# Autodesk Inventor assembly: Final
(part 2 of 3)
475. din1587-m5x0_8ricu3:15 — Mate:506, Mate:512
476. din1587-m5x0_8ricu3:16 — Mate:505, Mate:513
477. din1587-m5x0_8ricu3:17 — Mate:504, Mate:511
478. din1587-m6x1ricu3:3 — Mate:476, Mate:477
## Relationships (1050: Mate 990, Flush 53, Angle 7)
- Flush:1: bottom:1
- Flush:2: bottom:1
- Mate:1: bottom:1
- Mate:2: bottom:1 ↔ SeitenUntenHinten:1
- Mate:3: bottom:1 ↔ SeitenUntenHinten:1
- Mate:4: bottom:1 ↔ SeitenUntenHinten:1
- Mate:8: bottom:1 ↔ Heatsink:1
- Mate:9: bottom:1 ↔ Heatsink:1
- Mate:10: bottom:1 ↔ Heatsink:1
- Mate:11: EndStück_Caps:2 ↔ SeitenUntenHinten:1
- Mate:12: EndStück_Caps:2 ↔ SeitenUntenHinten:1
- Mate:13: EndStück_Caps:2 ↔ SeitenUntenHinten:1
- Mate:14: SeitenUntenHinten:1 ↔ Cap:1
- Mate:15: SeitenUntenHinten:1 ↔ Cap:2
- Mate:16: EndStück_Caps:2 ↔ Cap:2
- Mate:17: EndStück_Caps:2 ↔ Cap:1
- Mate:18: EndStück_Caps:1 ↔ Cap:1
- Mate:19: EndStück_Caps:1 ↔ Cap:1
- Mate:20: EndStück_Caps:1 ↔ Cap:2
- Mate:21: Cap:2 ↔ MidStück_Caps:1
- Mate:22: EndStück_Caps:1 ↔ MidStück_Caps:1
- Mate:23: Cap:1 ↔ MidStück_Caps:1
- Mate:24: SeitenUntenHinten:1 ↔ mid:1
- Mate:25: SeitenUntenHinten:1 ↔ mid:1
- Mate:26: SeitenUntenHinten:1 ↔ mid:1
- Mate:27: bottom:1 ↔ LogicHolder:1
- Mate:28: bottom:1 ↔ LogicHolder:1
- Mate:29: bottom:1 ↔ LogicHolder:1
- Mate:31: Elektronik_Gehäuse:1 ↔ LogicHolder:1
- Mate:32: Elektronik_Gehäuse:1 ↔ LogicHolder:1
- Mate:33: bottom:1 ↔ NtHolder:1
- Mate:36: bottom:1 ↔ SeitenUnten:2
- Mate:37: bottom:1 ↔ SeitenUnten:1
- Mate:38: bottom:1 ↔ SeitenUnten:1
- Mate:39: bottom:1 ↔ SeitenUnten:2
- Mate:40: bottom:1 ↔ SeitenUnten:2
- Mate:41: bottom:1 ↔ SeitenUnten:1
- Mate:42: SeitenUntenVorne:1 ↔ ToslinkHalter:1
- Mate:43: SeitenUntenVorne:1 ↔ ToslinkHalter:1
- Mate:45: Heatsink:1 ↔ GT175DA120U:2
- Mate:46: Heatsink:1 ↔ GT175DA120U:4
- Mate:47: Heatsink:1 ↔ GT175DA120U:3
- Mate:48: Heatsink:1 ↔ GT175DA120U:1
- Mate:49: Heatsink:1 ↔ GT175DA120U:1
- Mate:50: Heatsink:1 ↔ GT175DA120U:1
- Mate:51: Heatsink:1 ↔ GT175DA120U:2
- Mate:52: Heatsink:1 ↔ GT175DA120U:2
- Mate:53: Heatsink:1 ↔ GT175DA120U:4
- Mate:54: Heatsink:1 ↔ GT175DA120U:4
- Mate:55: Heatsink:1 ↔ GT175DA120U:3
- Mate:56: Heatsink:1 ↔ GT175DA120U:3
- Mate:57: IGBT_Platine:3 ↔ GT175DA120U:1
- Mate:58: IGBT_Platine:4 ↔ GT175DA120U:2
- Mate:59: IGBT_Platine:2 ↔ GT175DA120U:3
- Mate:60: IGBT_Platine:1 ↔ GT175DA120U:4
- Mate:61: IGBT_Platine:2 ↔ GT175DA120U:3
- Mate:62: IGBT_Platine:2 ↔ GT175DA120U:3
- Mate:63: IGBT_Platine:1 ↔ GT175DA120U:4
- Mate:64: IGBT_Platine:1 ↔ GT175DA120U:4
- Mate:65: IGBT_Platine:3 ↔ GT175DA120U:1
- Mate:66: IGBT_Platine:3 ↔ GT175DA120U:1
- Mate:67: IGBT_Platine:4 ↔ GT175DA120U:2
- Mate:68: IGBT_Platine:4 ↔ GT175DA120U:2
- Mate:69: IGBT_Platine:1 ↔ din125-1-a_4_3-140_hv:12
- Mate:70: IGBT_Platine:1 ↔ din125-1-a_4_3-140_hv:3
- Mate:71: IGBT_Platine:1 ↔ din125-1-a_4_3-140_hv:4
- Mate:72: IGBT_Platine:1 ↔ din125-1-a_4_3-140_hv:1
- Mate:73: IGBT_Platine:1 ↔ din125-1-a_4_3-140_hv:1
- Mate:74: IGBT_Platine:1 ↔ din125-1-a_4_3-140_hv:12
- Mate:75: IGBT_Platine:1 ↔ din125-1-a_4_3-140_hv:4
- Mate:76: IGBT_Platine:1 ↔ din125-1-a_4_3-140_hv:3
- Mate:77: Abstandshalter_12mm_M4:9 ↔ din125-1-a_4_3-140_hv:1
- Mate:78: Abstandshalter_12mm_M4:1 ↔ din125-1-a_4_3-140_hv:3
- Mate:79: Abstandshalter_12mm_M4:3 ↔ din125-1-a_4_3-140_hv:12
- Mate:80: GT175DA120U:4 ↔ Abstandshalter_12mm_M4:9
- Mate:81: GT175DA120U:4 ↔ Abstandshalter_12mm_M4:3
- Mate:82: GT175DA120U:4 ↔ Abstandshalter_12mm_M4:1
- Mate:83: IGBT_Platine:2 ↔ din125-1-a_4_3-140_hv:13
- Mate:84: IGBT_Platine:2 ↔ din125-1-a_4_3-140_hv:6
- Mate:85: IGBT_Platine:2 ↔ din125-1-a_4_3-140_hv:2
- Mate:86: IGBT_Platine:2 ↔ din125-1-a_4_3-140_hv:11
- Mate:87: IGBT_Platine:3 ↔ din125-1-a_4_3-140_hv:16
- Mate:88: IGBT_Platine:4 ↔ din125-1-a_4_3-140_hv:15
- Mate:89: IGBT_Platine:4 ↔ din125-1-a_4_3-140_hv:9
- Mate:90: IGBT_Platine:4 ↔ din125-1-a_4_3-140_hv:10
- Mate:91: IGBT_Platine:4 ↔ din125-1-a_4_3-140_hv:8
- Mate:92: IGBT_Platine:3 ↔ din125-1-a_4_3-140_hv:14
- Mate:93: IGBT_Platine:3 ↔ din125-1-a_4_3-140_hv:7
- Mate:94: IGBT_Platine:3 ↔ din125-1-a_4_3-140_hv:5
- Mate:95: GT175DA120U:1 ↔ din125-1-a_4_3-140_hv:7
- Mate:96: IGBT_Platine:3 ↔ din125-1-a_4_3-140_hv:5
- Mate:97: IGBT_Platine:3 ↔ din125-1-a_4_3-140_hv:14
- Mate:98: IGBT_Platine:3 ↔ din125-1-a_4_3-140_hv:16
- Mate:99: GT175DA120U:3 ↔ din125-1-a_4_3-140_hv:11
- Mate:100: GT175DA120U:3 ↔ din125-1-a_4_3-140_hv:6
- Mate:101: GT175DA120U:3 ↔ din125-1-a_4_3-140_hv:13
- Mate:102: GT175DA120U:3 ↔ din125-1-a_4_3-140_hv:2
- Mate:103: GT175DA120U:2 ↔ din125-1-a_4_3-140_hv:8
- Mate:104: GT175DA120U:2 ↔ din125-1-a_4_3-140_hv:10
- Mate:105: GT175DA120U:2 ↔ din125-1-a_4_3-140_hv:15
- Mate:106: GT175DA120U:2 ↔ din125-1-a_4_3-140_hv:9
- Mate:107: Abstandshalter_12mm_M4:2 ↔ din125-1-a_4_3-140_hv:8
- Mate:108: Abstandshalter_12mm_M4:4 ↔ din125-1-a_4_3-140_hv:9
- Mate:109: Abstandshalter_12mm_M4:6 ↔ din125-1-a_4_3-140_hv:15
- Mate:110: Abstandshalter_12mm_M4:5 ↔ din125-1-a_4_3-140_hv:5
- Mate:111: Abstandshalter_12mm_M4:7 ↔ din125-1-a_4_3-140_hv:14
- Mate:112: Abstandshalter_12mm_M4:15 ↔ din125-1-a_4_3-140_hv:7
- Mate:113: Abstandshalter_12mm_M4:16 ↔ din125-1-a_4_3-140_hv:13
- Mate:114: Abstandshalter_12mm_M4:8 ↔ din125-1-a_4_3-140_hv:6
- Mate:115: Abstandshalter_12mm_M4:10 ↔ din125-1-a_4_3-140_hv:11
- Mate:116: GT175DA120U:3 ↔ Abstandshalter_12mm_M4:16
- Mate:117: GT175DA120U:3 ↔ Abstandshalter_12mm_M4:8
- Mate:118: GT175DA120U:3 ↔ Abstandshalter_12mm_M4:10
- Mate:119: GT175DA120U:1 ↔ Abstandshalter_12mm_M4:7
- Mate:120: GT175DA120U:1 ↔ Abstandshalter_12mm_M4:15
- Mate:121: GT175DA120U:1 ↔ Abstandshalter_12mm_M4:5
- Mate:122: GT175DA120U:2 ↔ Abstandshalter_12mm_M4:6
- Mate:123: GT175DA120U:2 ↔ Abstandshalter_12mm_M4:4
- Mate:124: GT175DA120U:2 ↔ Abstandshalter_12mm_M4:2
- Mate:125: Abstandshalter_12mm_M4:7 ↔ CU6:1
- Mate:126: Abstandshalter_12mm_M4:15 ↔ CU6:1
- Mate:127: Abstandshalter_12mm_M4:7 ↔ CU6:1
- Mate:128: Abstandshalter_12mm_M4:3 ↔ CU5:1
- Mate:129: Abstandshalter_12mm_M4:16 ↔ CU5:1
- Mate:130: Abstandshalter_12mm_M4:9 ↔ CU5:1
- Mate:131: CU6:1 ↔ Snubber:1
- Mate:132: CU6:1 ↔ Snubber:1
- Mate:133: CU6:1 ↔ Snubber:2
- Mate:134: CU6:1 ↔ Snubber:2
- Mate:135: Abstandshalter_12mm_M4:1 ↔ CU7:1
- Mate:136: Abstandshalter_12mm_M4:1 ↔ CU7:1
- Mate:137: Abstandshalter_12mm_M4:2 ↔ CU7:1
- Mate:138: Snubber:3 ↔ CU7:1
- Mate:139: Snubber:4 ↔ CU7:1
- Mate:140: Snubber:3 ↔ CU7:1
- Mate:141: Snubber:4 ↔ CU7:1
- Mate:142: Abstandshalter_12mm_M4:5 ↔ CU8:1
- Mate:143: Abstandshalter_12mm_M4:5 ↔ CU8:1
- Mate:144: Abstandshalter_12mm_M4:4 ↔ CU8:1
- Mate:145: Snubber:2 ↔ CU8:1
- Mate:146: Snubber:4 ↔ CU8:1
- Mate:147: CU8:1 ↔ din_en_iso_4762_m4x6:6
- Mate:148: CU8:1 ↔ din_en_iso_4762_m4x6:4
- Mate:149: CU8:1 ↔ din_en_iso_4762_m4x6:2
- Mate:150: CU7:1 ↔ din_en_iso_4762_m4x6:5
- Mate:151: CU6:1 ↔ din_en_iso_4762_m4x6:8
- Mate:152: Abstandshalter_12mm_M4:7 ↔ din_en_iso_4762_m4x6:8
- Mate:153: Abstandshalter_12mm_M4:5 ↔ din_en_iso_4762_m4x6:2
- Mate:154: Abstandshalter_12mm_M4:4 ↔ din_en_iso_4762_m4x6:6
- Mate:155: Abstandshalter_12mm_M4:6 ↔ din_en_iso_4762_m4x6:4
- Mate:156: Abstandshalter_12mm_M4:2 ↔ din_en_iso_4762_m4x6:5
- Mate:157: Abstandshalter_12mm_M4:15 ↔ din_en_iso_4762_m4x6:1
- Mate:158: CU6:1 ↔ din_en_iso_4762_m4x6:1
- Mate:159: CU7:1 ↔ din_en_iso_4762_m4x6:7
- Mate:160: CU5:1 ↔ din_en_iso_4762_m4x6:9
- Mate:161: CU6:1 ↔ din_en_iso_4762_m4x6:3
- Mate:162: CU6:1 ↔ din_en_iso_4762_m4x6:10
- Mate:163: CU5:1 ↔ din_en_iso_4762_m4x6:11
- Mate:164: CU5:1 ↔ din_en_iso_4762_m4x6:12
- Mate:165: Abstandshalter_12mm_M4:1 ↔ din_en_iso_4762_m4x6:7
- Mate:166: Abstandshalter_12mm_M4:3 ↔ din_en_iso_4762_m4x6:9
- Mate:167: Abstandshalter_12mm_M4:8 ↔ din_en_iso_4762_m4x6:3
- Mate:168: Abstandshalter_12mm_M4:10 ↔ din_en_iso_4762_m4x6:10
- Mate:169: Abstandshalter_12mm_M4:16 ↔ din_en_iso_4762_m4x6:11
- Mate:170: Abstandshalter_12mm_M4:9 ↔ din_en_iso_4762_m4x6:12
- Mate:171: CU5:1 ↔ Snubber:1
- Mate:172: CU5:1 ↔ Snubber:3
- Mate:173: Snubber:4 ↔ din_en_iso_4762_m4x6:16
- Mate:174: Snubber:3 ↔ din_en_iso_4762_m4x6:15
- Mate:175: Snubber:2 ↔ din_en_iso_4762_m4x6:14
- Mate:176: Snubber:1 ↔ din_en_iso_4762_m4x6:13
- Mate:177: Snubber:2 ↔ din_en_iso_4762_m4x6:18
- Mate:178: Snubber:1 ↔ din_en_iso_4762_m4x6:17
- Mate:179: Snubber:4 ↔ din_en_iso_4762_m4x6:20
- Mate:180: Snubber:3 ↔ din_en_iso_4762_m4x6:19
- Mate:181: CU7:1 ↔ din_en_iso_4762_m4x6:15
- Mate:182: CU7:1 ↔ din_en_iso_4762_m4x6:16
- Mate:183: CU5:1 ↔ din_en_iso_4762_m4x6:13
- Mate:184: CU5:1 ↔ din_en_iso_4762_m4x6:19
- Mate:185: CU8:1 ↔ din_en_iso_4762_m4x6:20
- Mate:186: CU6:1 ↔ din_en_iso_4762_m4x6:17
- Mate:187: CU6:1 ↔ din_en_iso_4762_m4x6:18
- Mate:188: CU7:1 ↔ mutter_din934_m4-10:1
- Mate:189: CU7:1 ↔ mutter_din934_m4-10:2
- Mate:190: CU8:1 ↔ mutter_din934_m4-10:3
- Mate:191: CU8:1 ↔ mutter_din934_m4-10:4
- Mate:192: CU5:1 ↔ mutter_din934_m4-10:6
- Mate:193: din_en_iso_4762_m4x6:13 ↔ mutter_din934_m4-10:6
- Mate:194: din_en_iso_4762_m4x6:15 ↔ mutter_din934_m4-10:2
- Mate:195: din_en_iso_4762_m4x6:16 ↔ mutter_din934_m4-10:1
- Mate:196: din_en_iso_4762_m4x6:20 ↔ mutter_din934_m4-10:3
- Mate:197: din_en_iso_4762_m4x6:18 ↔ mutter_din934_m4-10:4
- Mate:198: CU5:1 ↔ mutter_din934_m4-10:5
- Mate:199: CU6:1 ↔ mutter_din934_m4-10:8
- Mate:200: CU8:1 ↔ mutter_din934_m4-10:7
- Mate:201: din_en_iso_4762_m4x6:14 ↔ mutter_din934_m4-10:7
- Mate:202: din_en_iso_4762_m4x6:19 ↔ mutter_din934_m4-10:5
- Mate:203: din_en_iso_4762_m4x6:17 ↔ mutter_din934_m4-10:8
- Mate:211: mid:1 ↔ Abstandshalter_10mm:3
- Mate:212: mid:1 ↔ Abstandshalter_10mm:2
- Mate:213: mid:1 ↔ Abstandshalter_10mm:4
- Mate:215: mid:1 ↔ Abstandshalter_10mm:17
- Mate:219: mid:1 ↔ Abstandshalter_10mm:8
- Mate:222: mid:1 ↔ Abstandshalter_10mm:19
- Mate:224: mid:1 ↔ Abstandshalter_10mm:9
- Mate:225: mid:1 ↔ Abstandshalter_10mm:11
- Mate:227: mid:1 ↔ Abstandshalter_10mm:19
- Mate:232: mid:1 ↔ Abstandshalter_10mm:3
- Mate:233: mid:1 ↔ Abstandshalter_10mm:4
- Mate:234: mid:1 ↔ Abstandshalter_10mm:2
- Mate:235: Abstandshalter_10mm:2 ↔ Cap_Platine:2
- Mate:242: Abstandshalter_10mm:3 ↔ Cap_Platine:1
- Mate:245: mid:1 ↔ Abstandshalter_10mm:7
- Mate:246: mid:1 ↔ Abstandshalter_10mm:7
- Mate:247: mid:1 ↔ Abstandshalter_10mm:9
- Mate:249: mid:1 ↔ Abstandshalter_10mm:17
- Mate:252: mid:1 ↔ Abstandshalter_10mm:14
- Mate:253: mid:1 ↔ Abstandshalter_10mm:14
- Mate:255: mid:1 ↔ Abstandshalter_10mm:11
- Mate:256: Abstandshalter_10mm:11 ↔ Cap_Platine:5
- Mate:259: mid:1 ↔ Abstandshalter_10mm:8
- Mate:260: Abstandshalter_10mm:8 ↔ Cap_Platine:4
- Mate:261: Abstandshalter_10mm:7 ↔ Cap_Platine:3
- Mate:268: mid:1 ↔ SeitenOben:3
- Mate:269: mid:1 ↔ SeitenOben:3
- Mate:270: mid:1 ↔ SeitenOben:1
- Mate:271: mid:1 ↔ SeitenOben:2
- Mate:272: mid:1 ↔ SeitenOben:4
- Mate:273: bottom:1 ↔ SeitenUntenVorne:1
- Mate:274: bottom:1 ↔ SeitenUntenVorne:1
- Mate:275: bottom:1 ↔ SeitenUntenVorne:1
- Mate:276: mid:1 ↔ SeitenOben:3
- Mate:277: mid:1 ↔ SeitenOben:2
- Mate:278: mid:1 ↔ SeitenOben:4
- Mate:279: mid:1 ↔ SeitenOben:1
- Mate:280: mid:1 ↔ SeitenOben:2
- Mate:281: mid:1 ↔ SeitenOben:4
- Mate:282: mid:1 ↔ SeitenOben:1
- Mate:283: Main:1 ↔ SeitenOben:4
- Mate:284: Main:1 ↔ SeitenOben:3
- Mate:285: Main:1 ↔ SeitenOben:2
- Mate:286: Main:1 ↔ M5 Gewindestange:2
- Mate:287: Main:1 ↔ M5 Gewindestange:3
- Mate:288: Main:1 ↔ M5 Gewindestange:1
- Mate:289: Main:1 ↔ M5 Gewindestange:4
- Flush:9 (-4 mm): bottom:1 ↔ M5 Gewindestange:3
- Flush:10 (4 mm): bottom:1 ↔ M5 Gewindestange:1
- Flush:11 (4 mm): bottom:1 ↔ M5 Gewindestange:2
- Flush:12 (4 mm): bottom:1 ↔ M5 Gewindestange:4
- Mate:290: Main:1 ↔ Seconday_End_Bottom:1
- Mate:291: Main:1 ↔ Seconday_End_Bottom:1
- Mate:292: PlexiHalter1:1 ↔ Seconday_End_Bottom:1
- Mate:293: PlexiHalter1:1 ↔ Seconday_End_Bottom:1
- Mate:296: M5 Gewindestange:4 ↔ mutter_din934_m5-6:7
- Mate:297: M5 Gewindestange:4 ↔ mutter_din934_m5-6:8
- Mate:298: M5 Gewindestange:1 ↔ mutter_din934_m5-6:6
- Mate:299: M5 Gewindestange:1 ↔ mutter_din934_m5-6:3
- Mate:300: M5 Gewindestange:2 ↔ mutter_din934_m5-6:4
- Mate:301: M5 Gewindestange:2 ↔ mutter_din934_m5-6:2
- Mate:302: M5 Gewindestange:3 ↔ mutter_din934_m5-6:1
- Mate:303: M5 Gewindestange:3 ↔ mutter_din934_m5-6:5
- Mate:304: Main:1 ↔ mutter_din934_m5-6:4
- Mate:305: Main:1 ↔ mutter_din934_m5-6:5
- Mate:306: Main:1 ↔ mutter_din934_m5-6:8
- Mate:307: Main:1 ↔ mutter_din934_m5-6:3
- Mate:308: mutter_din934_m5-6:6 ↔ Primary:1
- Mate:309: mutter_din934_m5-6:1 ↔ Primary:1
- Mate:310: mutter_din934_m5-6:7 ↔ Primary:1
- Mate:311: mutter_din934_m5-6:2 ↔ Primary:1
- Mate:312: bottom:1 ↔ din1587-m5x0_8ricu3:4
- Mate:313: bottom:1 ↔ din1587-m5x0_8ricu3:1
- Mate:314: bottom:1 ↔ din1587-m5x0_8ricu3:6
- Mate:315: bottom:1 ↔ din1587-m5x0_8ricu3:3
- Mate:316 (-4 mm): M5 Gewindestange:4 ↔ din1587-m5x0_8ricu3:2
- Mate:317 (-4 mm): M5 Gewindestange:2 ↔ din1587-m5x0_8ricu3:9
- Mate:318 (-4 mm): M5 Gewindestange:3 ↔ din1587-m5x0_8ricu3:5
- Mate:319 (-4 mm): M5 Gewindestange:1 ↔ din1587-m5x0_8ricu3:8
- Mate:320: M5 Gewindestange:2 ↔ din1587-m5x0_8ricu3:3
- Mate:321: M5 Gewindestange:3 ↔ din1587-m5x0_8ricu3:1
- Mate:322: M5 Gewindestange:4 ↔ din1587-m5x0_8ricu3:4
- Mate:323: M5 Gewindestange:1 ↔ din1587-m5x0_8ricu3:6
- Mate:324: M5 Gewindestange:1 ↔ din1587-m5x0_8ricu3:8
- Mate:325: M5 Gewindestange:4 ↔ din1587-m5x0_8ricu3:2
- Mate:326: M5 Gewindestange:2 ↔ din1587-m5x0_8ricu3:9
- Mate:327: M5 Gewindestange:3 ↔ din1587-m5x0_8ricu3:5
- Mate:328 (15 mm): Main:1 ↔ Primary:1
- Mate:329: Seconday_End_Bottom:1 ↔ mutter_din934_m6-6:1
- Mate:330: PlexiHalter1:1 ↔ Seconday_End_Bottom:1
- Mate:331: Seconday_End_Bottom:1 ↔ mutter_din934_m6-6:1
- Mate:332: PlexiHalter1:1 ↔ mutter_din934_m6-6:1
- Mate:333: PlexiHalter1:1 ↔ PlexiHalter2:2
- Mate:334: PlexiHalter1:1 ↔ PlexiHalter2:2
- Mate:335: PlexiHalter1:1 ↔ PlexiHalter2:2
- Mate:336: PlexiHalter2:2 ↔ din1587-m6x1ricu3:1
- Mate:337: PlexiHalter2:2 ↔ din1587-m6x1ricu3:1
- Mate:338: PlexiHalter1:2 ↔ Seconday_End_Top:1
- Mate:339: PlexiHalter1:2 ↔ Seconday_End_Top:1
- Mate:340: PlexiHalter1:2 ↔ PlexiHalter2:1
- Mate:341: Seconday_End_Top:1 ↔ mutter_din934_m6-6:2
- Mate:342: PlexiHalter1:2 ↔ mutter_din934_m6-6:2
- Mate:343: PlexiHalter1:2 ↔ Seconday_End_Top:1
- Mate:344: Seconday_End_Top:1 ↔ mutter_din934_m6-6:2
- Mate:345: PlexiHalter1:2 ↔ PlexiHalter2:1
- Mate:346: PlexiHalter1:2 ↔ PlexiHalter2:1
- Mate:347: PlexiHalter2:1 ↔ din1587-m6x1ricu3:2
- Mate:348: PlexiHalter2:1 ↔ din1587-m6x1ricu3:2
- Mate:349: Secondary:1 ↔ Coil:1
- Flush:13 (50 mm): Secondary:1 ↔ Coil:1
- Mate:350: Seconday_End_Bottom:1 ↔ Secondary:1
- Mate:351: Seconday_End_Top:1 ↔ Secondary:1
- Mate:352: Seconday_End_Bottom:1 ↔ Secondary:1
- Mate:353: Seconday_End_Top:1 ↔ Secondary:1
- Mate:354: Seconday_End_Top:1 ↔ M6 Gewindestange:1
- Mate:355: M6 Gewindestange:1 ↔ TopLoad:1
- Mate:356: Primary:1 ↔ primary_holder:6
- Mate:357: Primary:1 ↔ primary_holder:5
- Mate:358: Primary:1 ↔ primary_holder:1
- Mate:359: Primary:1 ↔ primary_holder:2
- Mate:360: Primary:1 ↔ primary_holder:4
- Mate:363: mid:1 ↔ din_en_iso_4762_m3x8:1
- Mate:366: M5 Gewindestange:4 ↔ Primary:1
- Mate:367: M5 Gewindestange:1 ↔ Primary:1
- Mate:368: Primary:1 ↔ primary_holder:3
- Mate:369: Primary:1 ↔ din_en_iso_4762_m4x12:1
- Mate:370: Primary:1 ↔ din_en_iso_4762_m4x12:4
- Mate:371: Primary:1 ↔ din_en_iso_4762_m4x12:2
- Mate:372: Primary:1 ↔ din_en_iso_4762_m4x12:3
- Mate:373: Primary:1 ↔ din_en_iso_4762_m4x12:2
- Mate:374: Primary:1 ↔ din_en_iso_4762_m4x12:1
- Mate:375: Primary:1 ↔ din_en_iso_4762_m4x12:4
- Mate:376: Primary:1 ↔ din_en_iso_4762_m4x12:3
- Mate:377: Primary:1 ↔ din_en_iso_4762_m4x12:12
- Mate:378: Primary:1 ↔ din_en_iso_4762_m4x12:11
- Mate:379: Primary:1 ↔ din_en_iso_4762_m4x12:9
- Mate:380: Primary:1 ↔ din_en_iso_4762_m4x12:7
- Mate:381: Primary:1 ↔ din_en_iso_4762_m4x12:10
- Mate:382: Primary:1 ↔ din_en_iso_4762_m4x12:8
- Mate:383: Primary:1 ↔ din_en_iso_4762_m4x12:6
- Mate:384: Primary:1 ↔ din_en_iso_4762_m4x12:5
- Mate:385: Primary:1 ↔ din_en_iso_4762_m4x12:10
- Mate:386: Primary:1 ↔ din_en_iso_4762_m4x12:8
- Mate:387: Primary:1 ↔ din_en_iso_4762_m4x12:9
- Mate:388: Primary:1 ↔ din_en_iso_4762_m4x12:12
- Mate:389: Primary:1 ↔ din_en_iso_4762_m4x12:5
- Mate:390: Primary:1 ↔ din_en_iso_4762_m4x12:7
- Mate:391: Primary:1 ↔ din_en_iso_4762_m4x12:6
- Mate:392: Primary:1 ↔ din_en_iso_4762_m4x12:11
- Mate:393: Secondary:1 ↔ din_en_iso_4762_m3x10:1
- Mate:394: Secondary:1 ↔ din_en_iso_4762_m3x10:2
- Mate:395: Secondary:1 ↔ din_en_iso_4762_m3x10:4
- Mate:396: Secondary:1 ↔ din_en_iso_4762_m3x10:3
- Mate:401: Secondary:1 ↔ din_en_iso_4762_m3x10:5
- Mate:402: Secondary:1 ↔ din_en_iso_4762_m3x10:6
- Mate:403: Secondary:1 ↔ din_en_iso_4762_m3x10:8
- Mate:404: Secondary:1 ↔ din_en_iso_4762_m3x10:7
- Mate:405: din_en_iso_4762_m3x10:1 ↔ mutter_din934_m3-6:4
- Mate:406: PlexiHalter1:2 ↔ mutter_din934_m3-6:4
- Mate:407 (-2 mm): din_en_iso_4762_m3x10:1 ↔ mutter_din934_m3-6:4
- Mate:408: din_en_iso_4762_m3x10:4 ↔ mutter_din934_m3-6:2
- Mate:409: din_en_iso_4762_m3x10:3 ↔ mutter_din934_m3-6:1
- Mate:410: din_en_iso_4762_m3x10:2 ↔ mutter_din934_m3-6:3
- Mate:411: PlexiHalter1:2 ↔ mutter_din934_m3-6:3
- Mate:412: PlexiHalter1:2 ↔ mutter_din934_m3-6:2
- Mate:413: PlexiHalter1:2 ↔ mutter_din934_m3-6:1
- Mate:414: PlexiHalter2:1 ↔ mutter_din934_m3-6:7
- Mate:415: PlexiHalter2:1 ↔ mutter_din934_m3-6:8
- Mate:416: PlexiHalter2:1 ↔ mutter_din934_m3-6:6
- Mate:417: PlexiHalter2:1 ↔ mutter_din934_m3-6:5
- Mate:422: din_en_iso_4762_m3x10:2 ↔ mutter_din934_m3-6:3
- Mate:423 (-2 mm): din_en_iso_4762_m3x10:3 ↔ mutter_din934_m3-6:1
- Mate:424 (-2 mm): din_en_iso_4762_m3x10:4 ↔ mutter_din934_m3-6:2
- Mate:425: PlexiHalter1:2 ↔ din_en_iso_7991_m3x16:1
- Mate:426: PlexiHalter1:2 ↔ din_en_iso_7991_m3x16:3
- Mate:427: PlexiHalter1:2 ↔ din_en_iso_7991_m3x16:2
- Mate:428: PlexiHalter1:2 ↔ din_en_iso_7991_m3x16:4
- Mate:429 (-3 mm): din1587-m6x1ricu3:2 ↔ M6 Gewindestange:1
- Mate:430 (150 mm): Seconday_End_Top:1 ↔ TopLoad:1
- Flush:432: Seconday_End_Top:1 ↔ din_en_iso_7991_m3x16:2
- Flush:14: Seconday_End_Top:1 ↔ din_en_iso_7991_m3x16:3
- Flush:15: Seconday_End_Top:1 ↔ din_en_iso_7991_m3x16:4
- Flush:16: Seconday_End_Top:1 ↔ din_en_iso_7991_m3x16:1
- Mate:431: din_en_iso_7991_m3x16:1 ↔ mutter_din934_m3-6:6
- Mate:432: din_en_iso_7991_m3x16:2 ↔ mutter_din934_m3-6:5
- Mate:433: din_en_iso_7991_m3x16:4 ↔ mutter_din934_m3-6:7
- Mate:434: din_en_iso_7991_m3x16:3 ↔ mutter_din934_m3-6:8
- Mate:435: M6 Gewindestange:1 ↔ top:1
- Flush:437 (150 mm): TopLoad:1 ↔ top:1
- Flush:438 (2.5 mm): primary_holder:3
- Mate:437 (-2.5 mm): primary_holder:5
- Mate:438: primary_holder:3 ↔ mutter_din934_m4-10:10
- Mate:439: din_en_iso_4762_m4x12:10 ↔ mutter_din934_m4-10:10
- Mate:440: primary_holder:3 ↔ mutter_din934_m4-10:9
- Mate:441: din_en_iso_4762_m4x12:11 ↔ mutter_din934_m4-10:9
- Mate:442: primary_holder:3 ↔ mutter_din934_m4-10:9
- Mate:443: primary_holder:3 ↔ mutter_din934_m4-10:10
- Mate:444: primary_holder:5 ↔ mutter_din934_m4-10:12
- Mate:445: primary_holder:5 ↔ mutter_din934_m4-10:11
- Mate:446: din_en_iso_4762_m4x12:12 ↔ mutter_din934_m4-10:11
- Mate:447: primary_holder:5 ↔ mutter_din934_m4-10:11
- Mate:448: din_en_iso_4762_m4x12:5 ↔ mutter_din934_m4-10:12
- Mate:449: primary_holder:5 ↔ mutter_din934_m4-10:12
- Mate:450: din_en_iso_4762_m4x12:8 ↔ mutter_din934_m4-10:13
- Mate:451: primary_holder:1 ↔ mutter_din934_m4-10:13
- Mate:452: primary_holder:1 ↔ mutter_din934_m4-10:14
- Mate:453: din_en_iso_4762_m4x12:9 ↔ mutter_din934_m4-10:14
- Mate:454: primary_holder:1 ↔ mutter_din934_m4-10:14
- Mate:455: primary_holder:1 ↔ mutter_din934_m4-10:13
- Mate:456: primary_holder:4 ↔ mutter_din934_m4-10:16
- Mate:457: din_en_iso_4762_m4x12:7 ↔ mutter_din934_m4-10:16
- Mate:458: CU8:1 ↔ din_en_iso_4762_m4x6:14
- Mate:459: primary_holder:4 ↔ mutter_din934_m4-10:16
- Mate:460: primary_holder:4 ↔ mutter_din934_m4-10:19
- Mate:461: din_en_iso_4762_m4x12:6 ↔ mutter_din934_m4-10:19
- Mate:462: primary_holder:6 ↔ mutter_din934_m4-10:20
- Mate:463: din_en_iso_4762_m4x12:4 ↔ mutter_din934_m4-10:20
- Mate:464: din_en_iso_4762_m4x12:3 ↔ mutter_din934_m4-10:17
- Mate:465: din_en_iso_4762_m4x12:2 ↔ mutter_din934_m4-10:18
- Mate:466: primary_holder:2 ↔ mutter_din934_m4-10:18
- Mate:467: primary_holder:2 ↔ mutter_din934_m4-10:17
- Mate:468: primary_holder:2 ↔ mutter_din934_m4-10:17
- Mate:469
- Angle:1 (30 deg)
- Mate:470
- Angle:2 (60 deg)
- Flush:472 (-2.5 mm): primary_holder:2
- Flush:473 (2.5 mm): primary_holder:4
- Flush:474 (2.5 mm): primary_holder:6
- Flush:475 (2.5 mm): primary_holder:1
- Mate:471: din_en_iso_4762_m4x12:1 ↔ mutter_din934_m4-10:15
- Mate:472: primary_holder:6 ↔ mutter_din934_m4-10:15
- Mate:473: primary_holder:6 ↔ mutter_din934_m4-10:15
- Mate:474: Secondary:1 ↔ Strike_Rail:1
- Mate:475: primary_holder:1 ↔ Strike_Rail:1
- Mate:476: Main:1 ↔ din1587-m6x1ricu3:3
- Mate:477: Main:1 ↔ din1587-m6x1ricu3:3
- Mate:478: NtHolder:1 ↔ mutter_din934_m4-10:21
- Mate:479: NtHolder:1 ↔ mutter_din934_m4-10:21
- Mate:480: bottom:1 ↔ mutter_din934_m4-10:21
- Mate:484: mid:1 ↔ din_en_iso_4762_m3x8:1
- Mate:485: LogicHolder:1 ↔ mutter_din934_m4-10:22
- Mate:486: LogicHolder:1 ↔ mutter_din934_m4-10:22
- Mate:487: bottom:1 ↔ mutter_din934_m4-10:22
- Mate:490: mid:1 ↔ Abstandshalter_10mm:28
- Mate:491: mid:1 ↔ Abstandshalter_10mm:25
- Mate:492: mid:1 ↔ Abstandshalter_10mm:28
- Mate:493: din_en_iso_4762_m3x8:1 ↔ Abstandshalter_10mm:25
- Mate:496: Abstandshalter_10mm:25 ↔ Cap_Platine:6
- Mate:497: Abstandshalter_10mm:28 ↔ Cap_Platine:6
- Mate:498: Abstandshalter_10mm:25 ↔ Cap_Platine:6
- Mate:499: EndStück_Caps:1 ↔ M5 Gewindestange_Cap:1
- Mate:500: EndStück_Caps:1 ↔ M5 Gewindestange_Cap:2
- Mate:501: EndStück_Caps:1 ↔ M5 Gewindestange_Cap:3
- Mate:502: EndStück_Caps:1 ↔ M5 Gewindestange_Cap:4
- Flush:476 (2.5 mm): EndStück_Caps:1 ↔ M5 Gewindestange_Cap:1
- Flush:477 (-2.5 mm): EndStück_Caps:1 ↔ M5 Gewindestange_Cap:3
- Flush:478 (2.5 mm): EndStück_Caps:1 ↔ M5 Gewindestange_Cap:2
- Flush:479 (-2.5 mm): EndStück_Caps:1 ↔ M5 Gewindestange_Cap:4
- Mate:503: EndStück_Caps:1 ↔ din1587-m5x0_8ricu3:14
- Mate:504: EndStück_Caps:1 ↔ din1587-m5x0_8ricu3:17
- Mate:505: EndStück_Caps:1 ↔ din1587-m5x0_8ricu3:16
- Mate:506: EndStück_Caps:1 ↔ din1587-m5x0_8ricu3:15
- Mate:507: EndStück_Caps:2 ↔ din1587-m5x0_8ricu3:11
- Mate:508: EndStück_Caps:2 ↔ din1587-m5x0_8ricu3:13
- Mate:509: EndStück_Caps:2 ↔ din1587-m5x0_8ricu3:12
- Mate:510: EndStück_Caps:2 ↔ din1587-m5x0_8ricu3:10
- Mate:511: M5 Gewindestange_Cap:4 ↔ din1587-m5x0_8ricu3:17
- Mate:512: M5 Gewindestange_Cap:2 ↔ din1587-m5x0_8ricu3:15
- Mate:513: M5 Gewindestange_Cap:1 ↔ din1587-m5x0_8ricu3:16
- Mate:514: M5 Gewindestange_Cap:3 ↔ din1587-m5x0_8ricu3:14
- Mate:515: M5 Gewindestange_Cap:3 ↔ din1587-m5x0_8ricu3:12
- Mate:516: M5 Gewindestange_Cap:1 ↔ din1587-m5x0_8ricu3:11
- Mate:517: M5 Gewindestange_Cap:2 ↔ din1587-m5x0_8ricu3:13
- Mate:518: M5 Gewindestange_Cap:4 ↔ din1587-m5x0_8ricu3:10
- Mate:519: Cap:2 ↔ Cu_Cap:1
- Mate:521: Cap:2 ↔ Cu_Cap:2
- Mate:523: Cap:1 ↔ Cu_Cap:1
- Mate:524: Cap:1 ↔ Cu_Cap:2
- Mate:525: Cu_Cap:2 ↔ din125-1-a_5_3-140_hv:4
- Mate:526: Cu_Cap:1 ↔ din125-1-a_5_3-140_hv:1
- Mate:527: Cu_Cap:2 ↔ din125-1-a_5_3-140_hv:2
- Mate:528: Cu_Cap:1 ↔ din125-1-a_5_3-140_hv:3
- Mate:529: Cu_Cap:2 ↔ din125-1-a_5_3-140_hv:4
- Mate:530: Cu_Cap:1 ↔ din125-1-a_5_3-140_hv:1
- Mate:531: Cu_Cap:1 ↔ din125-1-a_5_3-140_hv:3
- Mate:532: Cu_Cap:2 ↔ din125-1-a_5_3-140_hv:2
- Mate:533: Platine_Gleichrichter:1 ↔ din125-1-a_5_3-140_hv:4
- Mate:534: Platine_Gleichrichter:2 ↔ din125-1-a_5_3-140_hv:2
- Mate:535: Platine_Gleichrichter:1 ↔ din125-1-a_5_3-140_hv:1
- Mate:536: Platine_Gleichrichter:1 ↔ din125-1-a_5_3-140_hv:4
- Mate:537: Platine_Gleichrichter:2 ↔ din125-1-a_5_3-140_hv:2
- Mate:538: Platine_Gleichrichter:2 ↔ din125-1-a_5_3-140_hv:3
- Mate:539: din125-1-a_4_3-140_hv:10 ↔ din_en_iso_4762_m4x6:22
- Mate:540: din125-1-a_4_3-140_hv:10 ↔ din_en_iso_4762_m4x6:22
- Mate:541: din125-1-a_4_3-140_hv:4 ↔ din_en_iso_4762_m4x6:23
- Mate:542: din125-1-a_4_3-140_hv:2 ↔ din_en_iso_4762_m4x6:24
- Mate:543: din125-1-a_4_3-140_hv:16 ↔ din_en_iso_4762_m4x6:21
- Mate:544: din125-1-a_4_3-140_hv:16 ↔ din_en_iso_4762_m4x6:21
- Mate:545: din125-1-a_4_3-140_hv:2 ↔ din_en_iso_4762_m4x6:24
- Mate:546: din125-1-a_4_3-140_hv:4 ↔ din_en_iso_4762_m4x6:23
- [Mate]: PlexiHalter2:2 ↔ mutter_din934_m3-6:34
- [Mate]: din_en_iso_4762_m3x10:6 ↔ mutter_din934_m3-6:34
- [Mate]: din_en_iso_4762_m3x10:5 ↔ mutter_din934_m3-6:31
- [Mate]: PlexiHalter2:2 ↔ mutter_din934_m3-6:31
- [Mate]: din_en_iso_4762_m3x10:8 ↔ mutter_din934_m3-6:32
- [Mate]: PlexiHalter2:2 ↔ mutter_din934_m3-6:32
- [Mate]: din_en_iso_4762_m3x10:7 ↔ mutter_din934_m3-6:33
- [Mate]: PlexiHalter2:2 ↔ mutter_din934_m3-6:33
- [Mate]: PlexiHalter2:2 ↔ mutter_din934_m3-6:33
- [Mate]: PlexiHalter2:2 ↔ mutter_din934_m3-6:32
- [Mate]: PlexiHalter2:2 ↔ mutter_din934_m3-6:31
- [Mate]: PlexiHalter2:2 ↔ mutter_din934_m3-6:34
- [Mate] (-2 mm): din_en_iso_4762_m3x10:5 ↔ mutter_din934_m3-6:31
- [Mate] (-2 mm): din_en_iso_4762_m3x10:8 ↔ mutter_din934_m3-6:32
- [Mate] (-2 mm): din_en_iso_4762_m3x10:6 ↔ mutter_din934_m3-6:34
- [Mate] (-2 mm): din_en_iso_4762_m3x10:7 ↔ mutter_din934_m3-6:33
- Mate:563: mutter_din934_m6-6:1 ↔ M6 Gewindestange_Unten:1
- Mate:564 (-3 mm): din1587-m6x1ricu3:1 ↔ M6 Gewindestange_Unten:1
- Mate:565: Heatsink:1 ↔ Gleichrichter:1
- Mate:566: Heatsink:1 ↔ Gleichrichter:1
- Mate:570: SeitenUntenVorne:1 ↔ Schalter:1
- Mate:571: SeitenUntenVorne:1 ↔ Schalter:2
- Mate:572: SeitenUntenVorne:1 ↔ Schalter:1
- Mate:573: SeitenUntenVorne:1 ↔ Schalter:2
- Mate:574: bottom:1 ↔ din_en_iso_4762_m4x12:13
- Mate:575: bottom:1 ↔ din_en_iso_4762_m4x12:14
- Mate:576: bottom:1 ↔ din_en_iso_4762_m4x12:13
- Mate:577: bottom:1 ↔ din_en_iso_4762_m4x12:14
- Mate:586: SeitenUntenHinten:1 ↔ Netzstecker:1
- Mate:587: SeitenUntenHinten:1 ↔ Netzstecker:2
- Mate:588: SeitenUntenHinten:1 ↔ Netzstecker:2
- Mate:589: SeitenUntenHinten:1 ↔ Netzstecker:1
- Mate:590: SeitenUntenHinten:1 ↔ Netzstecker:1
- Mate:591: SeitenUntenHinten:1 ↔ Netzstecker:2
- Mate:593: Abstandshalter_10mm:17 ↔ Cap_Platine:4
- Mate:594: Abstandshalter_10mm:8 ↔ Cap_Platine:4
- Mate:595: Abstandshalter_10mm:4 ↔ Cap_Platine:2
- Mate:596: Abstandshalter_10mm:2 ↔ Cap_Platine:2
- Mate:597: Abstandshalter_10mm:19 ↔ Cap_Platine:1
- Mate:598: Abstandshalter_10mm:3 ↔ Cap_Platine:1
- Mate:599: Abstandshalter_10mm:7 ↔ Cap_Platine:3
- Mate:600: Abstandshalter_10mm:9 ↔ Cap_Platine:3
- Mate:601: Abstandshalter_10mm:14 ↔ Cap_Platine:5
- Mate:602: Abstandshalter_10mm:11 ↔ Cap_Platine:5
- Mate:603: mid:1 ↔ Abstandshalter_10mm:11
- Mate:604: mid:1 ↔ Abstandshalter_10mm:19
- Mate:605: mid:1 ↔ Abstandshalter_10mm:3
- Mate:606: mid:1 ↔ Abstandshalter_10mm:33
- Mate:607: mid:1 ↔ Abstandshalter_10mm:30
- Mate:608: mid:1 ↔ Abstandshalter_10mm:29
- Mate:609: mid:1 ↔ Abstandshalter_10mm:31
- Mate:610: mid:1 ↔ Abstandshalter_10mm:32
- Mate:611: mid:1 ↔ Abstandshalter_10mm:34
- Mate:612: mid:1 ↔ Abstandshalter_10mm:34
- Mate:613: mid:1 ↔ Abstandshalter_10mm:30
- Mate:614: mid:1 ↔ Abstandshalter_10mm:33
- Mate:615: mid:1 ↔ Abstandshalter_10mm:31
- Mate:616: mid:1 ↔ Abstandshalter_10mm:29
- Mate:617: mid:1 ↔ Abstandshalter_10mm:32
- Mate:618: Cap_Platine:3 ↔ Cap_CU_Oben:2
- Mate:619: Cap_Platine:3 ↔ Cap_CU_Oben:2
- Mate:620: Cap_Platine:6 ↔ Cap_CU_Oben:2
- Mate:621: Cap_Platine:4 ↔ Cap_CU_Oben:1
- Mate:622: Cap_Platine:4 ↔ Cap_CU_Oben:3
- Mate:623: Cap_Platine:5 ↔ Cap_CU_Oben:4
- Mate:624: Cap_Platine:5 ↔ Cap_CU_Oben:4
- Mate:625: Cap_Platine:1 ↔ Cap_CU_Oben:4
- Mate:626: Cap_Platine:4 ↔ Cap_CU_Oben:3
- Mate:627: Cap_Platine:4 ↔ Cap_CU_Oben:1
- Mate:628: Cap_Platine:6 ↔ Cap_CU_Oben:3
- Mate:629: Cap_Platine:1 ↔ Cap_CU_Oben:1
- Mate:630: Cap_Platine:5 ↔ Cap_CU_Oben:5
- Mate:631: Cap_Platine:5 ↔ Cap_CU_Oben:5
- Mate:632: Cap_Platine:2 ↔ Cap_CU_Oben:5
- Mate:633: Cap_Platine:6 ↔ mutter_din934_m6-6:3
- Mate:634: Cap_Platine:6 ↔ mutter_din934_m6-6:3
- Mate:635: Cap_Platine:6 ↔ mutter_din934_m6-6:9
- Mate:636: Cap_Platine:3 ↔ mutter_din934_m6-6:8
- Mate:637: Cap_Platine:3 ↔ mutter_din934_m6-6:11
- Mate:638: Cap_Platine:4 ↔ mutter_din934_m6-6:13
- Mate:640: Cap_Platine:4 ↔ mutter_din934_m6-6:4
- Mate:641: Cap_Platine:1 ↔ mutter_din934_m6-6:6
- Mate:642: Cap_Platine:1 ↔ mutter_din934_m6-6:7
- Mate:643: Cap_Platine:6 ↔ mutter_din934_m6-6:9
- Mate:644: Cap_Platine:1 ↔ mutter_din934_m6-6:7
- Mate:645: Cap_Platine:4 ↔ mutter_din934_m6-6:13
- Mate:646: Cap_Platine:3 ↔ mutter_din934_m6-6:8
- Mate:647: Cap_Platine:4 ↔ mutter_din934_m6-6:4
- Mate:648: Cap_Platine:3 ↔ mutter_din934_m6-6:11
- Mate:649: Cap_Platine:5 ↔ mutter_din934_m6-6:10
- Mate:650: Cap_Platine:5 ↔ mutter_din934_m6-6:14
- Mate:651: Cap_Platine:2 ↔ mutter_din934_m6-6:12
- Mate:652: Cap_Platine:5 ↔ mutter_din934_m6-6:10
- Mate:653: Cap_Platine:5 ↔ mutter_din934_m6-6:14
- Mate:654: Cap_Platine:2 ↔ mutter_din934_m6-6:12
- Mate:655: Cap_Platine:1 ↔ mutter_din934_m6-6:6
- Mate:656: Cap_Platine:2 ↔ mutter_din934_m6-6:5
- Mate:657: Cap_Platine:2 ↔ mutter_din934_m6-6:5
- Angle:3 (0 deg): SeitenUntenVorne:1 ↔ Schalter:1
- Angle:4 (0 deg): Schalter:1 ↔ Schalter:2
- Angle:5 (0 deg): Cap:1
- Angle:6 (0 deg): Heatsink:1 ↔ Gleichrichter:1
- Mate:658: Heatsink:1 ↔ mutter_din934_m3-6:10
- Mate:661: Heatsink:1 ↔ mutter_din934_m3-6:9
- Mate:664: Heatsink:1 ↔ mutter_din934_m3-6:11
- Mate:665: Heatsink:1 ↔ mutter_din934_m3-6:12
- Mate:666: bottom:1 ↔ din_en_iso_4762_m3x10:9
- Mate:667: bottom:1 ↔ din_en_iso_4762_m3x10:9
- Mate:668: bottom:1 ↔ din_en_iso_4762_m3x10:10
- Mate:669: bottom:1 ↔ din_en_iso_4762_m3x10:12
- Mate:670: bottom:1 ↔ din_en_iso_4762_m3x10:11
- Mate:671: bottom:1 ↔ din_en_iso_4762_m3x10:10
- Mate:672: bottom:1 ↔ din_en_iso_4762_m3x10:12
- Mate:673: bottom:1 ↔ din_en_iso_4762_m3x10:11
- Mate:674: SeitenUntenHinten:1 ↔ Netzfilter:1
- Mate:675: SeitenUntenHinten:1 ↔ Netzfilter:1
- Mate:676: SeitenUntenHinten:1 ↔ Netzfilter:1
- Mate:679: Cap_Platine:2 ↔ din_en_iso_4762_m6x10:10
- Mate:680: Cap_Platine:5 ↔ din_en_iso_4762_m6x10:3
- Mate:681: CU5:1 ↔ din_en_iso_4762_m6x10:4
- Mate:682: CU8:1 ↔ din_en_iso_4762_m6x10:2
- Mate:683: Cap_Platine:5 ↔ din_en_iso_4762_m6x10:9
- Mate:684: Cap_Platine:2 ↔ din_en_iso_4762_m6x10:1
- Mate:685: Cap_Platine:1 ↔ din_en_iso_4762_m6x10:5
- Mate:686: Cap_Platine:4 ↔ din_en_iso_4762_m6x10:8
- Mate:687: Cap_Platine:2 ↔ din_en_iso_4762_m6x10:10
- Mate:688: Cap_CU_Oben:5 ↔ din_en_iso_4762_m6x10:1
- Mate:689: Cap_CU_Oben:5 ↔ din_en_iso_4762_m6x10:3
- Mate:690: Cap_CU_Oben:4 ↔ din_en_iso_4762_m6x10:9
- Mate:691: Cap_Platine:4 ↔ din_en_iso_4762_m6x10:7
- Mate:692: Cap_Platine:1 ↔ din_en_iso_4762_m6x10:6
- Mate:693: Cap_CU_Oben:4 ↔ din_en_iso_4762_m6x10:5
- Mate:694: Cap_CU_Oben:1 ↔ din_en_iso_4762_m6x10:6
- Mate:695: Cap_CU_Oben:1 ↔ din_en_iso_4762_m6x10:8
- Mate:696: Cap_CU_Oben:3 ↔ din_en_iso_4762_m6x10:7
- Mate:697: mid:1 ↔ din_en_iso_4762_m3x8:11
- Mate:698: mid:1 ↔ din_en_iso_4762_m3x8:2
- Mate:699: GT175DA120U:2 ↔ din_en_iso_4762_m3x8:5
- Mate:700: GT175DA120U:4 ↔ din_en_iso_4762_m3x8:8
- Mate:701: GT175DA120U:4 ↔ din_en_iso_4762_m3x8:8
- Mate:702: GT175DA120U:2 ↔ din_en_iso_4762_m3x8:5
- Mate:703: GT175DA120U:3 ↔ din_en_iso_4762_m3x8:9
- Mate:704: GT175DA120U:3 ↔ din_en_iso_4762_m3x8:9
- Mate:705: GT175DA120U:1 ↔ din_en_iso_4762_m3x8:14
- Mate:706: mid:1 ↔ din_en_iso_4762_m3x8:15
- Mate:707: CU8:1 ↔ din_en_iso_4762_m6x10:2
- Mate:708: CU5:1 ↔ din_en_iso_4762_m6x10:4
- Mate:709: mid:1 ↔ din_en_iso_4762_m3x8:6
- Mate:710: mid:1 ↔ din_en_iso_4762_m3x8:13
- Mate:711: mid:1 ↔ din_en_iso_4762_m3x8:12
- Mate:712: mid:1 ↔ din_en_iso_4762_m3x8:3
- Mate:713: mid:1 ↔ din_en_iso_4762_m3x8:4
- Mate:714: mid:1 ↔ din_en_iso_4762_m3x8:10
- Mate:715: mid:1 ↔ din_en_iso_4762_m3x8:7
- Mate:716: mid:1 ↔ din_en_iso_4762_m3x8:7
- Mate:717: mid:1 ↔ din_en_iso_4762_m3x8:4
- Mate:718: mid:1 ↔ din_en_iso_4762_m3x8:10
- Mate:719: mid:1 ↔ din_en_iso_4762_m3x8:15
- Mate:720: mid:1 ↔ din_en_iso_4762_m3x8:2
- Mate:721: mid:1 ↔ din_en_iso_4762_m3x8:6
- Mate:722: mid:1 ↔ din_en_iso_4762_m3x8:13
- Mate:723: mid:1 ↔ din_en_iso_4762_m3x8:12
- Mate:724: mid:1 ↔ din_en_iso_4762_m3x8:19
- Mate:725: mid:1 ↔ din_en_iso_4762_m3x8:27
- Mate:726: GT175DA120U:3 ↔ din_en_iso_4762_m3x8:16
- Mate:727: GT175DA120U:4 ↔ din_en_iso_4762_m3x8:18
- Mate:728: GT175DA120U:3 ↔ din_en_iso_4762_m3x8:16
- Mate:729: GT175DA120U:4 ↔ din_en_iso_4762_m3x8:18
- Mate:730: GT175DA120U:2 ↔ din_en_iso_4762_m3x8:25
- Mate:731: GT175DA120U:1 ↔ din_en_iso_4762_m3x8:24
- Mate:732: GT175DA120U:2 ↔ din_en_iso_4762_m3x8:25
- Mate:733: GT175DA120U:1 ↔ din_en_iso_4762_m3x8:14
- Mate:734: GT175DA120U:1 ↔ din_en_iso_4762_m3x8:24
- Mate:735: mid:1 ↔ din_en_iso_4762_m3x8:26
- Mate:736: mid:1 ↔ din_en_iso_4762_m3x8:17
- Mate:737: mid:1 ↔ din_en_iso_4762_m3x8:21
- Mate:738: mid:1 ↔ din_en_iso_4762_m3x8:22
- Mate:741: mid:1 ↔ din_en_iso_4762_m3x8:11
- Mate:742: mid:1 ↔ din_en_iso_4762_m3x8:19
- Mate:743: mid:1 ↔ din_en_iso_4762_m3x8:22
- Mate:744: mid:1 ↔ din_en_iso_4762_m3x8:21
- Mate:745: mid:1 ↔ din_en_iso_4762_m3x8:17
- Mate:746: mid:1 ↔ din_en_iso_4762_m3x8:27
- Mate:747: mid:1 ↔ din_en_iso_4762_m3x8:26
- Mate:750: mid:1 ↔ din_en_iso_4762_m3x8:3
- Mate:751: din_en_iso_4762_m6x10:13 ↔ mutter_din934_m6-6:11
- Mate:752: din_en_iso_4762_m6x10:14 ↔ mutter_din934_m6-6:8
- Mate:753: din_en_iso_4762_m6x10:11 ↔ mutter_din934_m6-6:3
- Mate:754: din_en_iso_4762_m6x10:12 ↔ mutter_din934_m6-6:9
- Mate:755: Cap_Platine:3 ↔ din_en_iso_4762_m6x10:13
- Mate:756: Cap_CU_Oben:2 ↔ din_en_iso_4762_m6x10:14
- Mate:757: Cap_CU_Oben:2 ↔ din_en_iso_4762_m6x10:12
- Mate:758: Cap_CU_Oben:3 ↔ din_en_iso_4762_m6x10:11
- Mate:759: Platine_Gleichrichter:1 ↔ din_en_iso_4762_m5x10:4
- Mate:760: Platine_Gleichrichter:1 ↔ din_en_iso_4762_m5x10:2
- Mate:761: Cu_Cap:2 ↔ din_en_iso_4762_m5x10:3
- Mate:762: CU7:1 ↔ din_en_iso_4762_m5x10:1
- Mate:763: CU6:1 ↔ din_en_iso_4762_m5x10:6
- Mate:764: CU6:1 ↔ din_en_iso_4762_m5x10:6
- Mate:765: CU7:1 ↔ din_en_iso_4762_m5x10:1
- Mate:766: Cu_Cap:1 ↔ din_en_iso_4762_m5x10:7
- Mate:767: Platine_Gleichrichter:2 ↔ din_en_iso_4762_m5x10:8
- Mate:768: Platine_Gleichrichter:2 ↔ din_en_iso_4762_m5x10:5
- Mate:769: Platine_Gleichrichter:1 ↔ din_en_iso_4762_m5x10:2
- Mate:772: Platine_Gleichrichter:1 ↔ din_en_iso_4762_m5x10:4
- Mate:773: Platine_Gleichrichter:2 ↔ din_en_iso_4762_m5x10:8
- Mate:774: Platine_Gleichrichter:2 ↔ din_en_iso_4762_m5x10:5
- Mate:777: CU7:1 ↔ mutter_din934_m5-6:10
- Mate:778: din_en_iso_4762_m5x10:1 ↔ mutter_din934_m5-6:10
- Mate:779: CU6:1 ↔ mutter_din934_m5-6:9
- Mate:780: din_en_iso_4762_m5x10:6 ↔ mutter_din934_m5-6:9
- Mate:781: ToslinkHalter:1 ↔ din_en_iso_4762_m3x25:1
- Mate:782: ToslinkHalter:1 ↔ din_en_iso_4762_m3x25:2
- Mate:783: ToslinkHalter:1 ↔ din_en_iso_4762_m3x25:2
- Mate:784: ToslinkHalter:1 ↔ din_en_iso_4762_m3x25:1
- Mate:785: din_en_iso_4762_m3x25:2 ↔ mutter_din934_m3-6:19
- Mate:786: ToslinkHalter:1 ↔ mutter_din934_m3-6:19
- Mate:787: din_en_iso_4762_m3x25:2 ↔ mutter_din934_m3-6:17
- Mate:788: din_en_iso_4762_m3x25:2 ↔ mutter_din934_m3-6:13
- Mate:789: din_en_iso_4762_m3x25:1 ↔ mutter_din934_m3-6:20
- Mate:790: ToslinkHalter:1 ↔ mutter_din934_m3-6:20
- Mate:791: mutter_din934_m3-6:17 ↔ mutter_din934_m3-6:19
- Mate:792: mutter_din934_m3-6:13 ↔ mutter_din934_m3-6:17
- Mate:793: din_en_iso_4762_m3x25:2 ↔ mutter_din934_m3-6:14
- Mate:794: din_en_iso_4762_m3x25:1 ↔ mutter_din934_m3-6:18
- Mate:795: din_en_iso_4762_m3x25:1 ↔ mutter_din934_m3-6:16
- Mate:796: din_en_iso_4762_m3x25:1 ↔ mutter_din934_m3-6:15
- Mate:797: mutter_din934_m3-6:16 ↔ mutter_din934_m3-6:20
- Mate:798: mutter_din934_m3-6:16 ↔ mutter_din934_m3-6:18
- Mate:799: mutter_din934_m3-6:15 ↔ mutter_din934_m3-6:18
- Mate:800: mutter_din934_m3-6:13 ↔ mutter_din934_m3-6:14
- Mate:801: SeitenUntenVorne:1 ↔ mutter_din934_m3-6:14
- Mate:802: din_en_iso_4762_m3x25:2 ↔ mutter_din934_m3-6:22
- Mate:803: din_en_iso_4762_m3x25:1 ↔ mutter_din934_m3-6:21
- Mate:804: SeitenUntenVorne:1 ↔ mutter_din934_m3-6:21
- Mate:805: SeitenUntenVorne:1 ↔ mutter_din934_m3-6:22
- Mate:806: Cap_Platine:5 ↔ din_en_iso_4762_m3x6:9
- Mate:807: Cap_Platine:5 ↔ din_en_iso_4762_m3x6:6
- Mate:808: Cap_Platine:5 ↔ din_en_iso_4762_m3x6:1
- Mate:809: Cap_Platine:5 ↔ din_en_iso_4762_m3x6:6
- Mate:810: Cap_Platine:5 ↔ din_en_iso_4762_m3x6:9
- Mate:811: Cap_Platine:5 ↔ din_en_iso_4762_m3x6:1
- Mate:812: Cap_Platine:2 ↔ din_en_iso_4762_m3x6:10
- Mate:813: Cap_Platine:1 ↔ din_en_iso_4762_m3x6:18
- Mate:814: Cap_Platine:4 ↔ din_en_iso_4762_m3x6:16
- Mate:815: Cap_Platine:2 ↔ din_en_iso_4762_m3x6:17
- Mate:816: Cap_Platine:2 ↔ din_en_iso_4762_m3x6:15
- Mate:817: Cap_Platine:1 ↔ din_en_iso_4762_m3x6:14
- Mate:818: Cap_Platine:1 ↔ din_en_iso_4762_m3x6:7
- Mate:819: Cap_Platine:4 ↔ din_en_iso_4762_m3x6:12
- Mate:820: Cap_Platine:4 ↔ din_en_iso_4762_m3x6:4
- Mate:821: Cap_Platine:6 ↔ din_en_iso_4762_m3x6:3
- Mate:822: Cap_Platine:6 ↔ din_en_iso_4762_m3x6:2
- Mate:823: Cap_Platine:3 ↔ din_en_iso_4762_m3x6:13
- Mate:824: Cap_Platine:6 ↔ din_en_iso_4762_m3x6:11
- Mate:825: Cap_Platine:3 ↔ din_en_iso_4762_m3x6:5
- Mate:826: Cap_Platine:3 ↔ din_en_iso_4762_m3x6:8
- Mate:827: Cap_Platine:2 ↔ din_en_iso_4762_m3x6:10
- Mate:828: Cap_Platine:2 ↔ din_en_iso_4762_m3x6:15
- Mate:829: Cap_Platine:1 ↔ din_en_iso_4762_m3x6:14
- Mate:830: Cap_Platine:1 ↔ din_en_iso_4762_m3x6:7
- Mate:831: Cap_Platine:6 ↔ din_en_iso_4762_m3x6:3
- Mate:832: Cap_Platine:6 ↔ din_en_iso_4762_m3x6:2
- Mate:833: Cap_Platine:1 ↔ din_en_iso_4762_m3x6:18
- Mate:834: Cap_Platine:4 ↔ din_en_iso_4762_m3x6:16
- Mate:835: Cap_Platine:2 ↔ din_en_iso_4762_m3x6:17
- Mate:836: Cap_Platine:6 ↔ din_en_iso_4762_m3x6:11
- Mate:837: Cap_Platine:3 ↔ din_en_iso_4762_m3x6:13
- Mate:838: Cap_Platine:4 ↔ din_en_iso_4762_m3x6:12
- Mate:839: Cap_Platine:4 ↔ din_en_iso_4762_m3x6:4
- Mate:840: Cap_Platine:3 ↔ din_en_iso_4762_m3x6:8
- Mate:841: Cap_Platine:3 ↔ din_en_iso_4762_m3x6:5
- Mate:842: Secondary:1 ↔ PrimaryCoil:1
- Mate:843: primary_holder:6 ↔ PrimaryCoil:1
- Mate:844: SeitenUnten:2 ↔ Lüfter:4
- Mate:845: SeitenUnten:2 ↔ Lüfter:3